# Autodesk Inventor assembly: Cryostat top plate
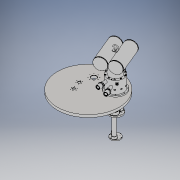
[picture p0: Inventor's stored thumbnail of the model, 180x180]
Saved by Autodesk Inventor 2018 (Build 220112000, 112)
## iProperties
Created: 2018-08-09
Part Number: Cryostat top plate
Document SubType Name: Assembly
Designer: QITI
Author: QITI
## Documents named in this file (3)
- C:\Users\QITI\Documents\Cryorefrigerator\CAD\Cryostat top plate.iam
- C:\Users\QITI\Documents\Cryorefrigerator\CAD\Top Plate.ipt
- C:\Users\QITI\Downloads\CH40415 24JUL14 C.ipt
## Components (2 placed, 2 different names)
1. Top Plate:1 — Mate:1, Mate:2, Mate:3
2. CH40415 24JUL14 C:1 — Mate:1, Mate:2, Mate:3
## Relationships (3: Mate 3)
- Mate:1: Top Plate:1 ↔ CH40415 24JUL14 C:1
- Mate:2: Top Plate:1 ↔ CH40415 24JUL14 C:1
- Mate:3: Top Plate:1 ↔ CH40415 24JUL14 C:1
